# Autodesk Inventor assembly: TopRoofAssemblyDrawing
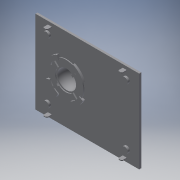
[picture p0: Inventor's stored thumbnail of the model, 180x180]
Saved by Autodesk Inventor 2017 (Build 210142000, 142)
## iProperties
Created: 2018-03-22
Part Number: TopRoofAssemblyDrawing
Document SubType Name: Assembly
Designer: Arjuna
Author: Arjuna
## Documents named in this file (4)
- D:\Users\Arjuna\Documents\NTU\FYP\Hardware\TopRoofAssemblyDrawing.iam
- D:\Users\Arjuna\Documents\NTU\FYP\Hardware\Top Roof.ipt
- D:\Users\Arjuna\Documents\NTU\FYP\Hardware\Dome Clip.ipt
- D:\Users\Arjuna\Documents\NTU\FYP\Hardware\Dome.ipt
## Components (3 placed, 3 different names)
1. Top Roof:1 — Insert:1, Insert:2
2. Dome Clip:1 — Insert:2
3. Dome:1 — Insert:1
## Relationships (2: Insert 2)
- Insert:1: Top Roof:1 ↔ Dome:1
- Insert:2: Top Roof:1 ↔ Dome Clip:1
